# Autodesk Inventor assembly: Assembly1
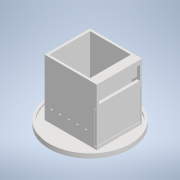
[picture p0: Inventor's stored thumbnail of the model, 180x180]
Saved by Autodesk Inventor 2022 (Build 260153000, 153)
## iProperties
Created: 2021-11-11
Part Number: Assembly1
Document SubType Name: Assembly
Designer: aed0019
Author: aed0019
## Documents named in this file (5)
- C:\Users\bonan\OneDrive\Desktop\Smarty Plants Files\Assembly1.iam
- C:\Users\bonan\OneDrive\Desktop\Smarty Plants Files\Drainage Base.ipt
- C:\Users\bonan\OneDrive\Desktop\Smarty Plants Files\SqPot.ipt
- C:\Users\bonan\OneDrive\Desktop\Smarty Plants Files\Door.ipt
- C:\Users\bonan\OneDrive\Desktop\Smarty Plants Files\Panel.ipt
## Components (4 placed, 4 different names)
1. Drainage Base:1
2. SqPot:1 — Mate:1, Mate:2, Flush:2
3. Door:1 — Mate:1, Mate:2
4. Panel:1 — Flush:2
## Relationships (3: Mate 2, Flush 1)
- Mate:1: SqPot:1 ↔ Door:1
- Mate:2: SqPot:1 ↔ Door:1
- Flush:2: SqPot:1 ↔ Panel:1
